# Autodesk Inventor assembly: CycloidalGear
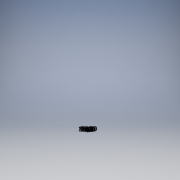
[picture p0: Inventor's stored thumbnail of the model, 180x180]
Saved by Autodesk Inventor 2018.3 (Build 223284000, 284)
## iProperties
Created: 2018-07-20
Part Number: CycloidalGear
Material: Generisch
Document SubType Name: Assembly
Designer: JochenAlt
Author: JochenAlt
## Documents named in this file (10)
- D:\Projects\FlowerPot\CAD\CycloidalGear\CycloidalGear.iam
- D:\Projects\FlowerPot\CAD\CycloidalGear\ExcentricShaft.ipt
- D:\Projects\FlowerPot\CAD\CycloidalGear\Excenter1.ipt
- D:\Projects\FlowerPot\CAD\CycloidalGear\Enclosure.ipt
- D:\Projects\FlowerPot\CAD\CycloidalGear\W 61701.iam
- D:\Projects\FlowerPot\CAD\CycloidalGear\Rotor.ipt
- C:\Users\JochenAlt\Documents\Inventor\Content Center Files\R2018\de-DE\BS 290 SKF(30)\BS 290 SKF - SKF 60_2.5.ipt
- D:\Projects\FlowerPot\CAD\CycloidalGear\Excenter2.ipt
- Excenter1.ipt
- D:\Projects\FlowerPot\CAD\CycloidalGear\ExcentricMotorShaft.ipt
## Components (21 placed, 7 different names)
1. Enclosure:1 — Passend:72, Fluchtend:19
2. W 61701:4 [sub-assembly]
3. W 61701:5 [sub-assembly] — Passend:15, Passend:26, Passend:29, Fluchtend:5, Passend:60, Fluchtend:10
4. ExcentricShaft:2 — Passend:62, Fluchtend:11, Passend:63, Fluchtend:12, Passend:74
5. ExcentricShaft:3 — Passend:15, Passend:26, Passend:29, Fluchtend:5, Passend:37, Passend:66, Passend:67, Passend:75
6. ExcentricShaft:4 — Passend:57, Fluchtend:8, Passend:73, -4, Fluchtend:21
7. Excenter1:2 — Passend:65, Passend:66, Fluchtend:15, Passend:70, Passend:76
8. W 61701:7 [sub-assembly] — Passend:63, Fluchtend:12, Passend:64, Fluchtend:13
9. W 61701:8 [sub-assembly] — Passend:57, Fluchtend:8, Passend:58, Fluchtend:14
10. W 61701:9 [sub-assembly] — Passend:37
11. W 61701:10 [sub-assembly] — Passend:62, Fluchtend:11, Passend:65
12. Rotor:1 — Passend:73, Passend:74, Passend:75, -4, Drehung:2
13. BS 290 SKF 60/2.5:1
14. BS 290 SKF 60/2.5:2
15. BS 290 SKF 60/2.5:3
16. Excenter1:3 — Passend:58, Passend:60, Fluchtend:10, Passend:64, Fluchtend:13, Fluchtend:14, Passend:71, Fluchtend:18, Drehung:1
17. MotorExcentricShaft:5 — Passend:54, Passend:55, Passend:61, Passend:68, Fluchtend:16, Passend:69, Fluchtend:17, Fluchtend:19, Drehung:1, Drehung:2
18. W 61701:11 [sub-assembly] — Passend:67, Fluchtend:15
19. W 61701:12 [sub-assembly] — Passend:68, Fluchtend:16, Passend:70
20. W 61701:13 [sub-assembly] — Passend:69, Fluchtend:17, Passend:71, Fluchtend:18
21. W 61701:14 [sub-assembly] — Passend:76, Fluchtend:21
## Relationships (41: Mate 25, Flush 14, RelateRotation 2)
- Passend:15 [Mate]: W 61701:5 ↔ ExcentricShaft:3
- Passend:26 [Mate]: W 61701:5 ↔ ExcentricShaft:3
- Passend:29 [Mate]: W 61701:5 ↔ ExcentricShaft:3
- Fluchtend:5 [Flush]: W 61701:5 ↔ ExcentricShaft:3
- Passend:37 [Mate]: ExcentricShaft:3 ↔ W 61701:9
- Passend:54 [Mate]: MotorExcentricShaft:5
- Passend:55 [Mate]: MotorExcentricShaft:5
- Passend:57 [Mate]: ExcentricShaft:4 ↔ W 61701:8
- Fluchtend:8 [Flush]: ExcentricShaft:4 ↔ W 61701:8
- Passend:58 [Mate]: W 61701:8 ↔ Excenter1:3
- Passend:60 [Mate]: W 61701:5 ↔ Excenter1:3
- Fluchtend:10 [Flush]: W 61701:5 ↔ Excenter1:3
- Passend:61 [Mate]: MotorExcentricShaft:5
- Passend:62 [Mate]: ExcentricShaft:2 ↔ W 61701:10
- Fluchtend:11 [Flush]: ExcentricShaft:2 ↔ W 61701:10
- Passend:63 [Mate]: ExcentricShaft:2 ↔ W 61701:7
- Fluchtend:12 [Flush]: ExcentricShaft:2 ↔ W 61701:7
- Passend:64 [Mate]: W 61701:7 ↔ Excenter1:3
- Fluchtend:13 [Flush]: W 61701:7 ↔ Excenter1:3
- Passend:65 [Mate]: Excenter1:2 ↔ W 61701:10
- Passend:66 [Mate]: ExcentricShaft:3 ↔ Excenter1:2
- Fluchtend:14 [Flush]: W 61701:8 ↔ Excenter1:3
- Passend:67 [Mate]: ExcentricShaft:3 ↔ W 61701:11
- Fluchtend:15 [Flush]: Excenter1:2 ↔ W 61701:11
- Passend:68 [Mate]: MotorExcentricShaft:5 ↔ W 61701:12
- Fluchtend:16 [Flush]: MotorExcentricShaft:5 ↔ W 61701:12
- Passend:69 [Mate]: MotorExcentricShaft:5 ↔ W 61701:13
- Fluchtend:17 [Flush]: MotorExcentricShaft:5 ↔ W 61701:13
- Passend:70 [Mate]: Excenter1:2 ↔ W 61701:12
- Passend:71 [Mate]: Excenter1:3 ↔ W 61701:13
- Fluchtend:18 [Flush]: Excenter1:3 ↔ W 61701:13
- Passend:72 [Mate]: Enclosure:1
- Fluchtend:19 [Flush]: Enclosure:1 ↔ MotorExcentricShaft:5
- Passend:73 [Mate]: ExcentricShaft:4 ↔ Rotor:1
- Passend:74 [Mate]: ExcentricShaft:2 ↔ Rotor:1
- Passend:75 [Mate]: ExcentricShaft:3 ↔ Rotor:1
- -4 [Flush] (-5 mm): ExcentricShaft:4 ↔ Rotor:1
- Drehung:1 [RelateRotation] (-0.1111 ul): Excenter1:3 ↔ MotorExcentricShaft:5
- Drehung:2 [RelateRotation] (0.1 ul): Rotor:1 ↔ MotorExcentricShaft:5
- Passend:76 [Mate]: Excenter1:2 ↔ W 61701:14
- Fluchtend:21 [Flush]: ExcentricShaft:4 ↔ W 61701:14
